# Autodesk Inventor assembly: CORL_000_CoralAssembly
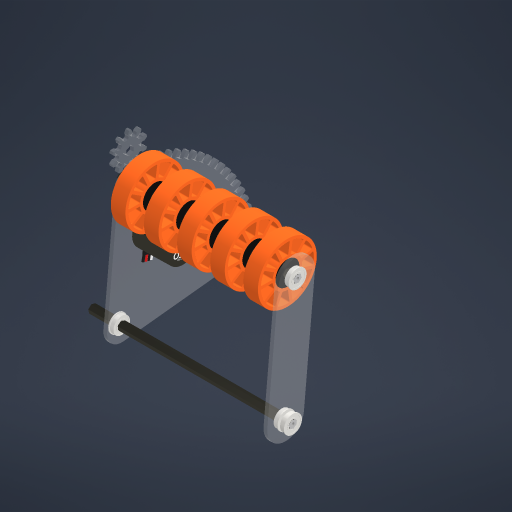
[picture p0: Inventor's stored thumbnail of the model, 512x512]
Saved by Autodesk Inventor 2024.2 (Build 282272000, 272)
## iProperties
Created: 2024-08-02
Part Number: CORL_000_CoralAssembly
Document SubType Name: Assembly
Designer: Bryan
Mass: 1860.11 g
Surface Area: 4686.68 cm^2
Volume: 1141.27 cm^3
Density: 1.62986 g/cm^3
Author: Bryan
## Documents named in this file (10)
- C:\Users\bobsb\OneDrive\Documents\GitHub\1622-2024-Summer-CAD-A-Thon\Coral\CORL_000_CoralAssembly.iam
- C:\Users\bobsb\OneDrive\Documents\GitHub\1622-2024-Summer-CAD-A-Thon\Coral\CORL_001_MainPlate.ipt
- C:\Users\bobsb\OneDrive\Documents\GitHub\1622-2024-Summer-CAD-A-Thon\COTS Library\Motion\Bearings\COTS_WCP-0783_1.125ODHexBearing.ipt
- C:\Users\bobsb\OneDrive\Documents\GitHub\1622-2024-Summer-CAD-A-Thon\Coral\CORL_002_FanPlate.ipt
- C:\Users\bobsb\OneDrive\Documents\GitHub\1622-2024-Summer-CAD-A-Thon\Coral\CORL_003_DropShaft.ipt
- C:\Users\bobsb\OneDrive\Documents\GitHub\1622-2024-Summer-CAD-A-Thon\Coral\CORL_004_PivotShaft.ipt
- C:\Users\bobsb\OneDrive\Documents\GitHub\1622-2024-Summer-CAD-A-Thon\Coral\CORL_005_PolyCarbSprocket.ipt
- C:\Users\bobsb\OneDrive\Documents\GitHub\1622-2024-Summer-CAD-A-Thon\COTS Library\Motion\Wheels\Compliant Wheels\4in compliant wheels\0.500in hex bore\COTS_am-3462_4indiameter_0.500inhexbore_durometer40A_CompliantWheel.ipt
- C:\Users\bobsb\OneDrive\Documents\GitHub\1622-2024-Summer-CAD-A-Thon\Coral\CORL_006_SmallPlate.ipt
- C:\Users\bobsb\OneDrive\Documents\GitHub\1622-2024-Summer-CAD-A-Thon\COTS Library\Motors\COTS_REV-21-1650-V1.1.ipt
## Components (27 placed, 9 different names)
1. CORL_001_MainPlate:1 — Mate:1, Mate:2, Mate:3, Mate:4, Mate:5, Mate:6, Mate:7, Mate:8, Mate:15, Mate:18, Mate:26, Mate:31, Flush:6
2. CORL_001_MainPlate:2 — Mate:1, Mate:2, Mate:3, Mate:9, Mate:10, Mate:11, Mate:12, Mate:13, Mate:29
3. COTS_WCP-0783_1.125ODHexBearing:1 — Mate:4
4. COTS_WCP-0783_1.125ODHexBearing:2 — Mate:5
5. COTS_WCP-0783_1.125ODHexBearing:3 — Mate:6
6. COTS_WCP-0783_1.125ODHexBearing:4 — Mate:7, Mate:26, Mate:30, Flush:2
7. COTS_WCP-0783_1.125ODHexBearing:5 — Mate:8
8. COTS_WCP-0783_1.125ODHexBearing:6 — Mate:9
9. COTS_WCP-0783_1.125ODHexBearing:7 — Mate:10, Mate:29
10. COTS_WCP-0783_1.125ODHexBearing:8 — Mate:11
11. COTS_WCP-0783_1.125ODHexBearing:9 — Mate:12
12. COTS_WCP-0783_1.125ODHexBearing:10 — Mate:13
13. CORL_002_FanPlate:2 — Mate:15, Mate:18, Mate:19, Mate:22, Mate:23, Mate:27, Flush:3, Mate:38, Mate:41, Mate:42, Mate:43, Tangent:2
14. COTS_WCP-0783_1.125ODHexBearing:11 — Mate:19, Mate:27
15. COTS_WCP-0783_1.125ODHexBearing:12 — Mate:33, Flush:5, Mate:36, Mate:37
16. COTS_WCP-0783_1.125ODHexBearing:13 — Mate:32, Flush:4, Flush:5, Mate:35
17. COTS_WCP-0783_1.125ODHexBearing:14 — Mate:22, Mate:23, Mate:25, Flush:1
18. CORL_003_DropShaft:1 — Mate:25, Flush:1, Mate:32, Flush:4, Mate:34
19. CORL_004_PivotShaft:1 — Mate:30, Flush:2, Mate:33
20. CORL_005_PolyCarbSprocket:1 — Mate:31, Flush:3, Tangent:2
21. CORL_006_SmallPlate:1 — Mate:35, Mate:36, Mate:37
22. COTS_REV-21-1650-V1.1:1 — Mate:41, Mate:42, Mate:43
23. COTS_am-3462_4indiameter_0.500inhexbore_durometer40A_CompliantWheel:1 — Mate:34, Tangent:1, Mate:38
24. COTS_am-3462_4indiameter_0.500inhexbore_durometer40A_CompliantWheel:2
25. COTS_am-3462_4indiameter_0.500inhexbore_durometer40A_CompliantWheel:3
26. COTS_am-3462_4indiameter_0.500inhexbore_durometer40A_CompliantWheel:4
27. COTS_am-3462_4indiameter_0.500inhexbore_durometer40A_CompliantWheel:5
## Component patterns: (5 elements, first: COTS_am-3462_4indiameter_0.500inhexbore_durometer40A_CompliantWheel:1)
## Relationships (42: Mate 34, Flush 6, Tangent 2)
- Mate:1: CORL_001_MainPlate:1 ↔ CORL_001_MainPlate:2
- Mate:2: CORL_001_MainPlate:1 ↔ CORL_001_MainPlate:2
- Mate:3 (333.375 mm): CORL_001_MainPlate:1 ↔ CORL_001_MainPlate:2
- Mate:4: CORL_001_MainPlate:1 ↔ COTS_WCP-0783_1.125ODHexBearing:1
- Mate:5: CORL_001_MainPlate:1 ↔ COTS_WCP-0783_1.125ODHexBearing:2
- Mate:6: CORL_001_MainPlate:1 ↔ COTS_WCP-0783_1.125ODHexBearing:3
- Mate:7: CORL_001_MainPlate:1 ↔ COTS_WCP-0783_1.125ODHexBearing:4
- Mate:8: CORL_001_MainPlate:1 ↔ COTS_WCP-0783_1.125ODHexBearing:5
- Mate:9: CORL_001_MainPlate:2 ↔ COTS_WCP-0783_1.125ODHexBearing:6
- Mate:10: CORL_001_MainPlate:2 ↔ COTS_WCP-0783_1.125ODHexBearing:7
- Mate:11: CORL_001_MainPlate:2 ↔ COTS_WCP-0783_1.125ODHexBearing:8
- Mate:12: CORL_001_MainPlate:2 ↔ COTS_WCP-0783_1.125ODHexBearing:9
- Mate:13: CORL_001_MainPlate:2 ↔ COTS_WCP-0783_1.125ODHexBearing:10
- Mate:15: CORL_001_MainPlate:1 ↔ CORL_002_FanPlate:2
- Mate:18 (38.1 mm): CORL_001_MainPlate:1 ↔ CORL_002_FanPlate:2
- Mate:19: CORL_002_FanPlate:2 ↔ COTS_WCP-0783_1.125ODHexBearing:11
- Mate:22: CORL_002_FanPlate:2 ↔ COTS_WCP-0783_1.125ODHexBearing:14
- Mate:23: CORL_002_FanPlate:2 ↔ COTS_WCP-0783_1.125ODHexBearing:14
- Mate:25: COTS_WCP-0783_1.125ODHexBearing:14 ↔ CORL_003_DropShaft:1
- Flush:1 (-12.7 mm): COTS_WCP-0783_1.125ODHexBearing:14 ↔ CORL_003_DropShaft:1
- Mate:26: CORL_001_MainPlate:1 ↔ COTS_WCP-0783_1.125ODHexBearing:4
- Mate:27: CORL_002_FanPlate:2 ↔ COTS_WCP-0783_1.125ODHexBearing:11
- Mate:29: CORL_001_MainPlate:2 ↔ COTS_WCP-0783_1.125ODHexBearing:7
- Mate:30: COTS_WCP-0783_1.125ODHexBearing:4 ↔ CORL_004_PivotShaft:1
- Flush:2: COTS_WCP-0783_1.125ODHexBearing:4 ↔ CORL_004_PivotShaft:1
- Mate:31: CORL_001_MainPlate:1 ↔ CORL_005_PolyCarbSprocket:1
- Flush:3: CORL_002_FanPlate:2 ↔ CORL_005_PolyCarbSprocket:1
- Mate:32: COTS_WCP-0783_1.125ODHexBearing:13 ↔ CORL_003_DropShaft:1
- Flush:4: COTS_WCP-0783_1.125ODHexBearing:13 ↔ CORL_003_DropShaft:1
- Mate:33: COTS_WCP-0783_1.125ODHexBearing:12 ↔ CORL_004_PivotShaft:1
- Flush:5: COTS_WCP-0783_1.125ODHexBearing:12 ↔ COTS_WCP-0783_1.125ODHexBearing:13
- Mate:34: CORL_003_DropShaft:1 ↔ COTS_am-3462_4indiameter_0.500inhexbore_durometer40A_CompliantWheel:1
- Flush:6 (31.75 mm): CORL_001_MainPlate:1
- Tangent:1: COTS_am-3462_4indiameter_0.500inhexbore_durometer40A_CompliantWheel:1
- Mate:35: COTS_WCP-0783_1.125ODHexBearing:13 ↔ CORL_006_SmallPlate:1
- Mate:36: COTS_WCP-0783_1.125ODHexBearing:12 ↔ CORL_006_SmallPlate:1
- Mate:37: COTS_WCP-0783_1.125ODHexBearing:12 ↔ CORL_006_SmallPlate:1
- Mate:38 (12.7 mm): CORL_002_FanPlate:2 ↔ COTS_am-3462_4indiameter_0.500inhexbore_durometer40A_CompliantWheel:1
- Mate:41: CORL_002_FanPlate:2 ↔ COTS_REV-21-1650-V1.1:1
- Mate:42: CORL_002_FanPlate:2 ↔ COTS_REV-21-1650-V1.1:1
- Mate:43: CORL_002_FanPlate:2 ↔ COTS_REV-21-1650-V1.1:1
- Tangent:2: CORL_002_FanPlate:2 ↔ CORL_005_PolyCarbSprocket:1
